# Autodesk Inventor assembly: Link6
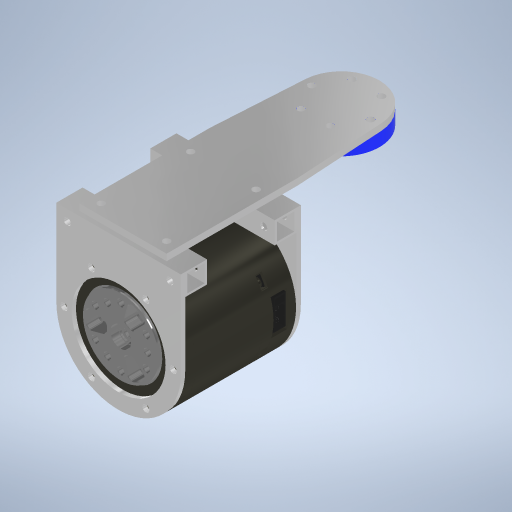
[picture p0: Inventor's stored thumbnail of the model, 512x512]
Saved by Autodesk Inventor 2024 (Build 280153000, 153)
## iProperties
Created: 2024-12-13
Part Number: Link6
Document SubType Name: Assembly
Designer: hirek
Mass: 381.567 g
Surface Area: 776.395 cm^2
Volume: 68.2473 cm^3
Density: 5.59095 g/cm^3
Author: hirek
## Documents named in this file (7)
- E:\Documents\Inventor\CanAloha\Link6.iam
- E:\Documents\Inventor\CanAloha\official\robStride00\robStride00.iam
- E:\Documents\Inventor\CanAloha\myperts\link4_plate2.ipt
- E:\Documents\Inventor\CanAloha\myperts\link4_plate3.ipt
- E:\Documents\Inventor\CanAloha\myperts\link4_pipe1.ipt
- E:\Documents\Inventor\CanAloha\myperts\link6_plate1.ipt
- E:\Documents\Inventor\CanAloha\myperts\link5_plate1.ipt
## Components (7 placed, 6 different names)
1. robStride00:1 [sub-assembly] — 回転:11, 回転:12, 回転:13, 回転:14
2. link4_plate2:1 — 回転:11, 回転:12, 回転:15, 回転:16
3. link4_plate3:1 — 回転:13, 回転:14, 回転:17, 回転:18
4. link4_pipe1:1 — 回転:15, 回転:16, 回転:20
5. link4_pipe1:2 — 回転:17, 回転:18, 回転:19
6. link6_plate1:1 — 回転:19, 回転:20, 回転:21, 回転:22
7. link5_plate1:1 — 回転:21, 回転:22
## Relationships (12: RevoluteJoint 12)
- 回転:11 [RevoluteJoint]: robStride00:1 ↔ link4_plate2:1
- 回転:12 [RevoluteJoint]: robStride00:1 ↔ link4_plate2:1
- 回転:13 [RevoluteJoint]: robStride00:1 ↔ link4_plate3:1
- 回転:14 [RevoluteJoint]: robStride00:1 ↔ link4_plate3:1
- 回転:15 [RevoluteJoint]: link4_plate2:1 ↔ link4_pipe1:1
- 回転:16 [RevoluteJoint]: link4_plate2:1 ↔ link4_pipe1:1
- 回転:17 [RevoluteJoint]: link4_plate3:1 ↔ link4_pipe1:2
- 回転:18 [RevoluteJoint]: link4_plate3:1 ↔ link4_pipe1:2
- 回転:19 [RevoluteJoint]: link4_pipe1:2 ↔ link6_plate1:1
- 回転:20 [RevoluteJoint]: link4_pipe1:1 ↔ link6_plate1:1
- 回転:21 [RevoluteJoint]: link6_plate1:1 ↔ link5_plate1:1
- 回転:22 [RevoluteJoint]: link6_plate1:1 ↔ link5_plate1:1
